# Autodesk Inventor assembly: DisplayModuleAssembly
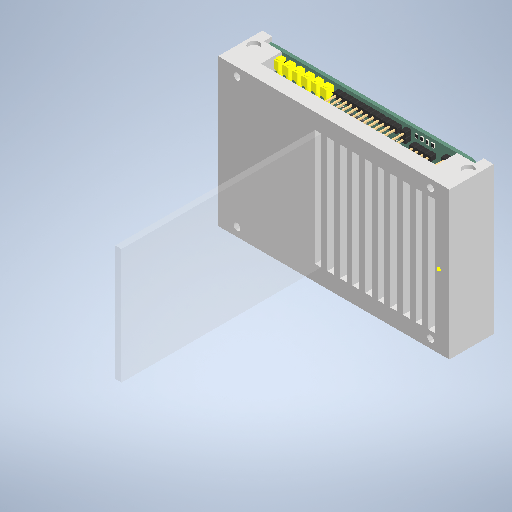
[picture p0: Inventor's stored thumbnail of the model, 512x512]
Saved by Autodesk Inventor 2025.1 (Build 291241020, 241B)
## iProperties
Created: 2024-09-25
Part Number: DisplayModuleAssembly
Document SubType Name: Assembly
Designer: Si Teng Wu
Author: Si Teng Wu
## Documents named in this file (4)
- C:\Users\Si Teng Wu\OneDrive - University of Cape Town\2024\EEE4022S\IOT_Retro_Display_EEE4022S\3D Models\DisplayModuleAssembly.iam
- C:\Users\Si Teng Wu\OneDrive - University of Cape Town\2024\EEE4022S\IOT_Retro_Display_EEE4022S\3D Models\DisplayModule.ipt
- C:\Users\Si Teng Wu\OneDrive - University of Cape Town\2024\EEE4022S\IOT_Retro_Display_EEE4022S\3D Models\DisplayModuleHousing.ipt
- C:\Users\Si Teng Wu\OneDrive - University of Cape Town\2024\EEE4022S\IOT_Retro_Display_EEE4022S\3D Models\AcrylicPane.ipt
## Components (3 placed, 3 different names)
1. DisplayModule:1 — Mate:6, Mate:7, Flush:1
2. DisplayModuleHousing:1 — Mate:6, Mate:7, Flush:1, Mate:8, Mate:9, Mate:10
3. AcrylicPane:1 — Mate:8, Mate:9, Mate:10
## Relationships (6: Mate 5, Flush 1)
- Mate:6 (0.25 mm): DisplayModule:1 ↔ DisplayModuleHousing:1
- Mate:7: DisplayModule:1 ↔ DisplayModuleHousing:1
- Flush:1: DisplayModule:1 ↔ DisplayModuleHousing:1
- Mate:8: DisplayModuleHousing:1 ↔ AcrylicPane:1
- Mate:9 (0.1 mm): DisplayModuleHousing:1 ↔ AcrylicPane:1
- Mate:10 (0.1 mm): DisplayModuleHousing:1 ↔ AcrylicPane:1
